# Autodesk Inventor assembly: test fit
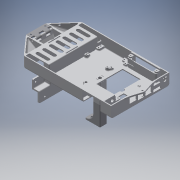
[picture p0: Inventor's stored thumbnail of the model, 180x180]
Saved by Autodesk Inventor 2019 (Build 230136000, 136)
## iProperties
Created: 2020-12-01
Part Number: test fit
Document SubType Name: Assembly
Designer: close
Author: close
## Documents named in this file (6)
- C:\Users\infinity\Documents\GitHub\barc_hardware\Enclosure\Nano&XAVIER\V_2\test fit.iam
- C:\Users\infinity\Documents\GitHub\barc_hardware\Enclosure\Nano&XAVIER\V_2\Enclosure_Dual_v2.ipt
- C:\Users\infinity\Documents\GitHub\barc_hardware\Enclosure\Nano&XAVIER\V_2\hinge_v1.ipt
- C:\Users\infinity\Documents\GitHub\barc_hardware\Enclosure\Nano&XAVIER\V_2\Camera Mount 43mm_all.ipt
- C:\Users\infinity\Documents\GitHub\barc_hardware\Enclosure\Nano&XAVIER\V_2\Dual Camera Mount.ipt
- C:\Users\infinity\Documents\GitHub\barc_hardware\Enclosure\Nano&XAVIER\V_2\vive_mount.ipt
## Components (6 placed, 5 different names)
1. Enclosure_Dual_v2:1 — Insert:1, Insert:2, Insert:3
2. hinge_v1:1 — Insert:1
3. Camera Mount 43mm_all:1 — Insert:2, Insert:5
4. Camera Mount 43mm_all:2 — Insert:3, Insert:4
5. Dual Camera Mount:1 — Insert:4
6. vive_mount:1 — Insert:5
## Relationships (5: Insert 5)
- Insert:1 (9.8 mm): Enclosure_Dual_v2:1 ↔ hinge_v1:1
- Insert:2: Enclosure_Dual_v2:1 ↔ Camera Mount 43mm_all:1
- Insert:3: Enclosure_Dual_v2:1 ↔ Camera Mount 43mm_all:2
- Insert:4: Camera Mount 43mm_all:2 ↔ Dual Camera Mount:1
- Insert:5: Camera Mount 43mm_all:1 ↔ vive_mount:1
